# Autodesk Inventor assembly: TraditionalWaterBathAssemblyNA11
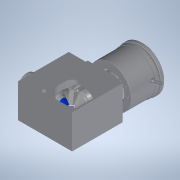
[picture p0: Inventor's stored thumbnail of the model, 180x180]
Saved by Autodesk Inventor 2022 (Build 260153000, 153)
## iProperties
Created: 2016-01-12
Part Number: TraditionalWaterBathAssemblyNA11
Document SubType Name: Assembly
Designer: 120pa
Author: 120pa
## Documents named in this file (9)
- C:\Users\Spectral\Documents\GitHub\CAD\Manuscripts\Isogai-2021\NA1pt1-Chamber-Assembly.iam
- C:\Users\Spectral\Documents\GitHub\CAD\Manuscripts\Isogai-2021\ChamberV4.ipt
- C:\Users\Spectral\Documents\GitHub\CAD\components\Nikon\N25XW-Apo-LWD-NA1pt1.ipt
- C:\Users\Spectral\Documents\GitHub\CAD\Manuscripts\Isogai-2021\Chamber-Plate-NA11.ipt
- C:\Users\Spectral\Documents\GitHub\CAD\Manuscripts\Isogai-2021\NA1pt1-Piezo-Extension.ipt
- C:\Users\Spectral\Documents\GitHub\CAD\components\PhysikInstrumente\P-726.1CD.ipt
- C:\Users\Spectral\Documents\GitHub\CAD\Manuscripts\Isogai-2021\Chamber-Plate-Circle.ipt
- C:\Users\Spectral\Documents\GitHub\CAD\Manuscripts\Isogai-2021\Collagen-Tension-Mount.ipt
- C:\Users\Spectral\Documents\GitHub\CAD\components\SpecialOptics\54-10-7.ipt
## Components (8 placed, 8 different names)
1. ChamberV4:1 — Mate:2, Mate:23, Angle:1, Mate:26, Mate:27, Mate:28, Mate:33, Angle:3
2. N25XW-Apo-LWD-NA1pt1:2 — Mate:2, Mate:29, Mate:30, Mate:32, Mate:34
3. Chamber-Plate-NA11:1 — Mate:26, Mate:27, Mate:28
4. NA1pt1-Piezo-Extension:1 — Mate:29, Mate:30, Mate:31
5. P-726.1CD:1 — Mate:31, Mate:32
6. Chamber-Plate-Circle:1 — Mate:23
7. Collagen-Tension-Mount:1 — Angle:1, Angle:3
8. 54-10-7:1 — Mate:33, Mate:34
## Relationships (13: Mate 11, Angle 2)
- Mate:2: ChamberV4:1 ↔ N25XW-Apo-LWD-NA1pt1:2
- Mate:23: ChamberV4:1 ↔ Chamber-Plate-Circle:1
- Angle:1 (0 deg): ChamberV4:1 ↔ Collagen-Tension-Mount:1
- Mate:26: ChamberV4:1 ↔ Chamber-Plate-NA11:1
- Mate:27: ChamberV4:1 ↔ Chamber-Plate-NA11:1
- Mate:28: ChamberV4:1 ↔ Chamber-Plate-NA11:1
- Mate:29: N25XW-Apo-LWD-NA1pt1:2 ↔ NA1pt1-Piezo-Extension:1
- Mate:30: N25XW-Apo-LWD-NA1pt1:2 ↔ NA1pt1-Piezo-Extension:1
- Mate:31: NA1pt1-Piezo-Extension:1 ↔ P-726.1CD:1
- Mate:32: N25XW-Apo-LWD-NA1pt1:2 ↔ P-726.1CD:1
- Mate:33: ChamberV4:1 ↔ 54-10-7:1
- Mate:34 (6.74 mm): N25XW-Apo-LWD-NA1pt1:2 ↔ 54-10-7:1
- Angle:3 (0 deg): ChamberV4:1 ↔ Collagen-Tension-Mount:1
